# Autodesk Inventor assembly: TestAssembly
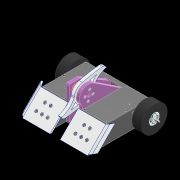
[picture p0: Inventor's stored thumbnail of the model, 180x180]
Saved by Autodesk Inventor 2021 (Build 250183000, 183)
## iProperties
Created: 2020-10-21
Part Number: TestAssembly
Document SubType Name: Assembly
Designer: Esketitttttt
Mass: 292.669 g
Surface Area: 1602.77 cm^2
Volume: 313.709 cm^3
Density: 0.932931 g/cm^3
Author: Esketitttttt
## Documents named in this file (13)
- C:\Users\Esketitttttt\Documents\GrabCAD\Insomnia 2020\RRW\TestAssembly.iam
- C:\Users\Esketitttttt\Documents\GrabCAD\Insomnia 2020\RRW\Chasis.ipt
- C:\Users\Esketitttttt\Documents\GrabCAD\Insomnia 2020\RRW\4-40 x 0.375_ flat head (0.148g).ipt
- C:\Users\Esketitttttt\Documents\GrabCAD\Insomnia 2020\RRW\FingerTech_Silver_Spark_223350.ipt
- C:\Users\Esketitttttt\Documents\GrabCAD\Insomnia 2020\RRW\Twist_Hub_4mmx075.ipt
- C:\Users\Esketitttttt\Documents\GrabCAD\Insomnia 2020\RRW\2_56 Thread_ 3_8 in Long_BUTTON HEAD HEX DRIVE SCREW.ipt
- C:\Users\Esketitttttt\Documents\GrabCAD\Insomnia 2020\RRW\WeaponAssembly.iam
- C:\Users\Esketitttttt\Documents\GrabCAD\Insomnia 2020\RRW\power switch _1_.iam
- C:\Users\Esketitttttt\Documents\GrabCAD\Insomnia 2020\RRW\2-56 x 0.5_ SHCS (0.146g).ipt
- C:\Users\Esketitttttt\Documents\GrabCAD\Insomnia 2020\RRW\2-56 locknut (0.778g) _1_.iam
- C:\Users\Esketitttttt\Documents\GrabCAD\Insomnia 2020\RRW\TopPlate.ipt
- C:\Users\Esketitttttt\Documents\GrabCAD\Insomnia 2020\RRW\MetalFrontRightWedge.ipt
- C:\Users\Esketitttttt\Documents\GrabCAD\Insomnia 2020\RRW\MetalFrontLeftWedge.ipt
## Components (40 placed, 12 different names)
1. Chasis:1 — Insert:9, Insert:10, Insert:11, Insert:12, Insert:29, Insert:30, Insert:47, Insert:48, Insert:49, Insert:50, Insert:51, Insert:52, Insert:53, Insert:54, Insert:55, Insert:56, Insert:57, Insert:58, Insert:80, Insert:81, Insert:92, Insert:93, Insert:94, Insert:95
2. FingerTech_Silver_Spark_223350:1 — Insert:9, Insert:10
3. FingerTech_Silver_Spark_223350:2 — Insert:11, Insert:12
4. MetalFrontRightWedge:1 — Insert:92, Insert:93, Insert:96, Insert:97, Insert:98, Insert:99, Insert:100
5. MetalFrontLeftWedge:1 — Insert:94, Insert:95, Insert:101, Insert:102, Insert:103, Insert:104, Insert:105
6. Twist_Hub_4mmx075:1 — Insert:29
7. Twist_Hub_4mmx075:2 — Insert:30
8. WeaponAssembly:1 [sub-assembly] — Insert:47, Insert:48
9. power switch _1_:1 [sub-assembly] — Insert:55, Insert:56, Insert:59, Insert:60
10. TopPlate:1 — Insert:80, Insert:81, Insert:82, Insert:83, Insert:84, Insert:85, Insert:86, Insert:87, Insert:88, Insert:89, Insert:90, Insert:91
11. 4-40 x 0.375_ flat head (0.148g):7 — Insert:104
12. 4-40 x 0.375_ flat head (0.148g):8 — Insert:105
13. 4-40 x 0.375_ flat head (0.148g):9 — Insert:101
14. 4-40 x 0.375_ flat head (0.148g):10 — Insert:102
15. 4-40 x 0.375_ flat head (0.148g):11 — Insert:103
16. 4-40 x 0.375_ flat head (0.148g):12 — Insert:100
17. 4-40 x 0.375_ flat head (0.148g):13 — Insert:99
18. 4-40 x 0.375_ flat head (0.148g):14 — Insert:98
19. 4-40 x 0.375_ flat head (0.148g):15 — Insert:96
20. 4-40 x 0.375_ flat head (0.148g):16 — Insert:97
21. 4-40 x 0.375_ flat head (0.148g):1 — Insert:54
22. 4-40 x 0.375_ flat head (0.148g):2 — Insert:52
23. 4-40 x 0.375_ flat head (0.148g):3 — Insert:53
24. 4-40 x 0.375_ flat head (0.148g):4 — Insert:49
25. 4-40 x 0.375_ flat head (0.148g):5 — Insert:50
26. 4-40 x 0.375_ flat head (0.148g):6 — Insert:51
27. 2-56 x 0.5_ SHCS (0.146g):1 — Insert:58
28. 2-56 x 0.5_ SHCS (0.146g):2 — Insert:57
29. 2-56 locknut (0.778g) _1_:1 [sub-assembly] — Insert:60
30. 2-56 locknut (0.778g) _1_:2 [sub-assembly] — Insert:59
31. 2_56 Thread_ 3_8 in Long_BUTTON HEAD HEX DRIVE SCREW:13 — Insert:87
32. 2_56 Thread_ 3_8 in Long_BUTTON HEAD HEX DRIVE SCREW:14 — Insert:88
33. 2_56 Thread_ 3_8 in Long_BUTTON HEAD HEX DRIVE SCREW:15 — Insert:90
34. 2_56 Thread_ 3_8 in Long_BUTTON HEAD HEX DRIVE SCREW:16 — Insert:89
35. 2_56 Thread_ 3_8 in Long_BUTTON HEAD HEX DRIVE SCREW:17 — Insert:91
36. 2_56 Thread_ 3_8 in Long_BUTTON HEAD HEX DRIVE SCREW:18 — Insert:85
37. 2_56 Thread_ 3_8 in Long_BUTTON HEAD HEX DRIVE SCREW:19 — Insert:82
38. 2_56 Thread_ 3_8 in Long_BUTTON HEAD HEX DRIVE SCREW:20 — Insert:83
39. 2_56 Thread_ 3_8 in Long_BUTTON HEAD HEX DRIVE SCREW:21 — Insert:84
40. 2_56 Thread_ 3_8 in Long_BUTTON HEAD HEX DRIVE SCREW:22 — Insert:86
## Relationships (46: Insert 46)
- Insert:9: Chasis:1 ↔ FingerTech_Silver_Spark_223350:1
- Insert:10: Chasis:1 ↔ FingerTech_Silver_Spark_223350:1
- Insert:11: Chasis:1 ↔ FingerTech_Silver_Spark_223350:2
- Insert:12: Chasis:1 ↔ FingerTech_Silver_Spark_223350:2
- Insert:29 (3.81 mm): Chasis:1 ↔ Twist_Hub_4mmx075:1
- Insert:30 (3.81 mm): Chasis:1 ↔ Twist_Hub_4mmx075:2
- Insert:47: Chasis:1 ↔ WeaponAssembly:1
- Insert:48: Chasis:1 ↔ WeaponAssembly:1
- Insert:49: Chasis:1 ↔ 4-40 x 0.375_ flat head (0.148g):4
- Insert:50: Chasis:1 ↔ 4-40 x 0.375_ flat head (0.148g):5
- Insert:51: Chasis:1 ↔ 4-40 x 0.375_ flat head (0.148g):6
- Insert:52: Chasis:1 ↔ 4-40 x 0.375_ flat head (0.148g):2
- Insert:53: Chasis:1 ↔ 4-40 x 0.375_ flat head (0.148g):3
- Insert:54: Chasis:1 ↔ 4-40 x 0.375_ flat head (0.148g):1
- Insert:55: Chasis:1 ↔ power switch _1_:1
- Insert:56: Chasis:1 ↔ power switch _1_:1
- Insert:57: Chasis:1 ↔ 2-56 x 0.5_ SHCS (0.146g):2
- Insert:58: Chasis:1 ↔ 2-56 x 0.5_ SHCS (0.146g):1
- Insert:59: power switch _1_:1 ↔ 2-56 locknut (0.778g) _1_:2
- Insert:60: power switch _1_:1 ↔ 2-56 locknut (0.778g) _1_:1
- Insert:80: Chasis:1 ↔ TopPlate:1
- Insert:81: Chasis:1 ↔ TopPlate:1
- Insert:82: TopPlate:1 ↔ 2_56 Thread_ 3_8 in Long_BUTTON HEAD HEX DRIVE SCREW:19
- Insert:83: TopPlate:1 ↔ 2_56 Thread_ 3_8 in Long_BUTTON HEAD HEX DRIVE SCREW:20
- Insert:84: TopPlate:1 ↔ 2_56 Thread_ 3_8 in Long_BUTTON HEAD HEX DRIVE SCREW:21
- Insert:85: TopPlate:1 ↔ 2_56 Thread_ 3_8 in Long_BUTTON HEAD HEX DRIVE SCREW:18
- Insert:86: TopPlate:1 ↔ 2_56 Thread_ 3_8 in Long_BUTTON HEAD HEX DRIVE SCREW:22
- Insert:87: TopPlate:1 ↔ 2_56 Thread_ 3_8 in Long_BUTTON HEAD HEX DRIVE SCREW:13
- Insert:88: TopPlate:1 ↔ 2_56 Thread_ 3_8 in Long_BUTTON HEAD HEX DRIVE SCREW:14
- Insert:89: TopPlate:1 ↔ 2_56 Thread_ 3_8 in Long_BUTTON HEAD HEX DRIVE SCREW:16
- Insert:90: TopPlate:1 ↔ 2_56 Thread_ 3_8 in Long_BUTTON HEAD HEX DRIVE SCREW:15
- Insert:91: TopPlate:1 ↔ 2_56 Thread_ 3_8 in Long_BUTTON HEAD HEX DRIVE SCREW:17
- Insert:92: Chasis:1 ↔ MetalFrontRightWedge:1
- Insert:93: Chasis:1 ↔ MetalFrontRightWedge:1
- Insert:94: Chasis:1 ↔ MetalFrontLeftWedge:1
- Insert:95: Chasis:1 ↔ MetalFrontLeftWedge:1
- Insert:96: MetalFrontRightWedge:1 ↔ 4-40 x 0.375_ flat head (0.148g):15
- Insert:97: MetalFrontRightWedge:1 ↔ 4-40 x 0.375_ flat head (0.148g):16
- Insert:98: MetalFrontRightWedge:1 ↔ 4-40 x 0.375_ flat head (0.148g):14
- Insert:99: MetalFrontRightWedge:1 ↔ 4-40 x 0.375_ flat head (0.148g):13
- Insert:100: MetalFrontRightWedge:1 ↔ 4-40 x 0.375_ flat head (0.148g):12
- Insert:101: MetalFrontLeftWedge:1 ↔ 4-40 x 0.375_ flat head (0.148g):9
- Insert:102: MetalFrontLeftWedge:1 ↔ 4-40 x 0.375_ flat head (0.148g):10
- Insert:103: MetalFrontLeftWedge:1 ↔ 4-40 x 0.375_ flat head (0.148g):11
- Insert:104: MetalFrontLeftWedge:1 ↔ 4-40 x 0.375_ flat head (0.148g):7
- Insert:105: MetalFrontLeftWedge:1 ↔ 4-40 x 0.375_ flat head (0.148g):8
